# Autodesk Inventor assembly: Complete Assembly
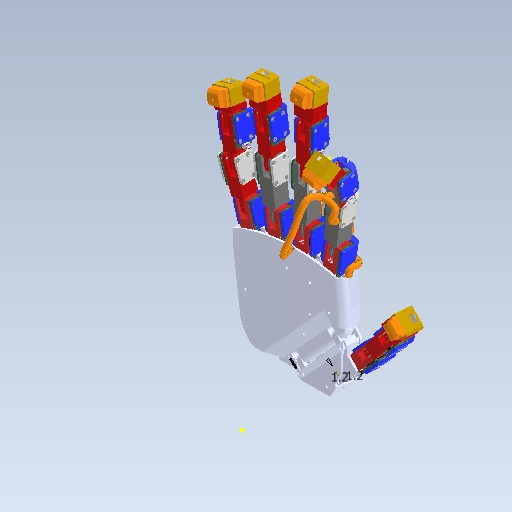
[picture p0: Inventor's stored thumbnail of the model, 512x512]
Saved by Autodesk Inventor 2020 (Build 240168000, 168)
## iProperties
Created: 2020-02-06
Part Number: Complete Assembly
Document SubType Name: Assembly
Designer: ttail
Sending System: SolidWorks 2018
Last Author: ttail
Last Saved: 2020-02-06
Author: ttail
## Documents named in this file (9)
- C:\Users\sami_\Documents\V1.6\Workgroups\NotInProject\Complete Assembly.iam
- C:\Users\sami_\Documents\V1.6\Workgroups\NotInProject\RING\finger RING.iam
- C:\Users\sami_\Documents\V1.6\Workgroups\NotInProject\INDEX\finger INDEX.iam
- C:\Users\sami_\Documents\V1.6\Workgroups\NotInProject\THUMB\Assembly\Complete Thumb.iam
- C:\Users\sami_\Documents\V1.6\Workgroups\NotInProject\PINKY\finger PINKY.iam
- C:\Users\sami_\Documents\V1.6\Workgroups\NotInProject\MIDDLE\finger MIDDLE.iam
- C:\Users\sami_\Documents\V1.6\Workgroups\NotInProject\Palm\FullCircularAssembly.iam
- C:\Users\sami_\Documents\V1.6\thumbL1.iam
- C:\Users\sami_\Documents\V1.6\Workgroups\NotInProject\Complete Assembly\AIP\Tube and Pipe\Cable and Harness\Complete Assembly.Harness5.iam
## Components (8 placed, 8 different names)
1. finger RING:1 [sub-assembly]
2. finger MIDDLE:1 [sub-assembly]
3. finger INDEX:1 [sub-assembly]
4. Complete Thumb:1 [sub-assembly]
5. finger PINKY:1 [sub-assembly]
6. FullCircularAssembly:1 [sub-assembly] — Mate:86
7. thumbL1:1 [sub-assembly]
8. Harness5 [sub-assembly]
## Relationships (17: Mate 8, WeldJoint 7, RevoluteJoint 2)
- [WeldJoint]: finger INDEX:1 ↔ FullCircularAssembly:1
- [WeldJoint]: finger PINKY:1 ↔ FullCircularAssembly:1
- [WeldJoint]: finger MIDDLE:1 ↔ FullCircularAssembly:1
- [RevoluteJoint]: Complete Thumb:1 ↔ thumbL1:1
- [WeldJoint]: finger RING:1 ↔ FullCircularAssembly:1
- Mate:86: FullCircularAssembly:1
- [Mate]: finger PINKY:1 ↔ FullCircularAssembly:1
- [Mate]: finger RING:1 ↔ FullCircularAssembly:1
- [Mate]: finger MIDDLE:1 ↔ FullCircularAssembly:1
- [Mate]: finger INDEX:1 ↔ FullCircularAssembly:1
- [Mate]: FullCircularAssembly:1 ↔ thumbL1:1
- [Mate]: FullCircularAssembly:1 ↔ thumbL1:1
- [WeldJoint]: FullCircularAssembly:1 ↔ thumbL1:1
- [RevoluteJoint]: FullCircularAssembly:1 ↔ thumbL1:1
- [WeldJoint]: FullCircularAssembly:1 ↔ thumbL1:1
- [WeldJoint]: FullCircularAssembly:1 ↔ thumbL1:1
- [Mate]: FullCircularAssembly:1 ↔ thumbL1:1
